# Autodesk Inventor assembly: BrandschutzAssemlby
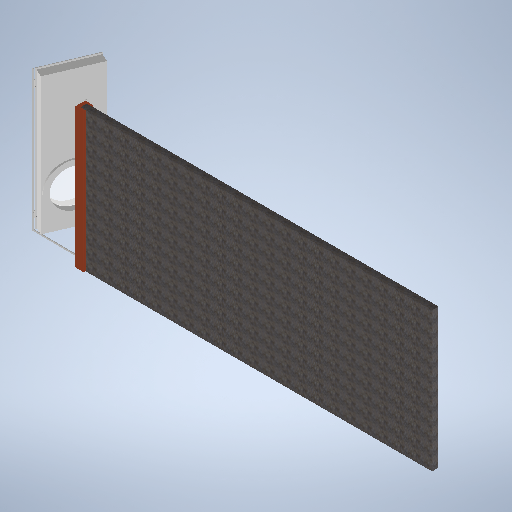
[picture p0: Inventor's stored thumbnail of the model, 512x512]
Saved by Autodesk Inventor 2025.1 (Build 291241000, 241)
## iProperties
Created: 2024-08-07
Part Number: BrandschutzAssemlby
Document SubType Name: Assembly
Designer: ffogue
Author: ffogue
## Documents named in this file (7)
- C:\Users\ffogue\Documents\Inventor\BrandschutzTuer\BrandschutzAssemlby.iam
- C:\Users\ffogue\Documents\Inventor\BrandschutzTuer\Wand.ipt
- C:\Users\ffogue\Documents\Inventor\BrandschutzTuer\ZargeRahmen.ipt
- C:\Users\ffogue\Documents\Inventor\BrandschutzTuer\Dichtung.iam
- C:\Users\ffogue\Documents\Inventor\BrandschutzTuer\Tuer.iam
- C:\Users\ffogue\Documents\Inventor\BrandschutzTuer\verbindungunten.ipt
- C:\Users\ffogue\Documents\Inventor\BrandschutzTuer\verbindung2.ipt
## Components (10 placed, 6 different names)
1. Wand:1 — Flush:1, Mate:1
2. ZargeRahmen:1 — Flush:1, Mate:1, Flush:2
3. Dichtung:1 [sub-assembly] — Flush:2, Mate:5, Mate:6, Mate:9, Mate:10, Insert:5
4. Tuer:1 [sub-assembly] — Mate:2, Insert:1, Mate:3, Insert:2, Mate:7, Mate:8, Insert:3, Insert:4
5. verbindungunten:1 — Mate:2, Insert:1, Rotational:1
6. verbindungunten:2 — Mate:3, Insert:2
7. verbindung2:1 — Rotational:1, Mate:5, Mate:6
8. verbindungunten:3 — Mate:7, Insert:3, Rotational:2
9. verbindungunten:4 — Mate:8, Insert:4, Mate:11
10. verbindung2:2 — Rotational:2, Mate:9, Mate:10, Mate:11, Insert:5
## Relationships (19: Mate 10, Insert 5, Flush 2, RevoluteJoint 2)
- Flush:1: Wand:1 ↔ ZargeRahmen:1
- Mate:1: Wand:1 ↔ ZargeRahmen:1
- Mate:2: Tuer:1 ↔ verbindungunten:1
- Insert:1 (-15 mm): Tuer:1 ↔ verbindungunten:1
- Mate:3: Tuer:1 ↔ verbindungunten:2
- Insert:2 (-15 mm): Tuer:1 ↔ verbindungunten:2
- Flush:2: ZargeRahmen:1 ↔ Dichtung:1
- Rotational:1 [RevoluteJoint] (8 mm): verbindungunten:1 ↔ verbindung2:1
- Mate:5: Dichtung:1 ↔ verbindung2:1
- Mate:6: Dichtung:1 ↔ verbindung2:1
- Mate:7: Tuer:1 ↔ verbindungunten:3
- Mate:8: Tuer:1 ↔ verbindungunten:4
- Insert:3 (-15 mm): Tuer:1 ↔ verbindungunten:3
- Insert:4 (-15 mm): Tuer:1 ↔ verbindungunten:4
- Rotational:2 [RevoluteJoint] (8 mm): verbindungunten:3 ↔ verbindung2:2
- Mate:9: Dichtung:1 ↔ verbindung2:2
- Mate:10: Dichtung:1 ↔ verbindung2:2
- Mate:11: verbindungunten:4 ↔ verbindung2:2
- Insert:5 (-13 mm): Dichtung:1 ↔ verbindung2:2
